# Autodesk Inventor assembly: one side of drive
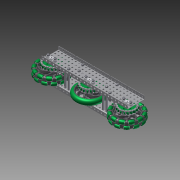
[picture p0: Inventor's stored thumbnail of the model, 180x180]
Saved by Autodesk Inventor 2014 SP1 (Build 180222100, 222)
## iProperties
Created: 2013-08-29
Part Number: one side of drive
Document SubType Name: Assembly
Designer: Ryan
Sending System: SolidWorks 2013
Last Author: Ryan
Author: Ryan
## Documents named in this file (15)
- C:\Users\Ryan\Desktop\sw\toss up 1st A bot\inventor drive\one side of drive.iam
- C:\Users\Ryan\Desktop\sw\lib\Aperture VEX CAD Library\Metal\C Channel\5 x 25.ipt
- C:\Users\Ryan\Desktop\sw\lib\Aperture VEX CAD Library\Bearing Blocks\Bearing Block.ipt
- C:\Users\Ryan\Desktop\sw\lib\Aperture VEX CAD Library\Shaft\2 inch Shaft.ipt
- C:\Users\Ryan\Desktop\sw\toss up 1st A bot\inventor drive\tensioner.iam
- C:\Users\Ryan\Desktop\sw\lib\Aperture VEX CAD Library\Standoffs\BEAM-2000.ipt
- C:\Users\Ryan\Desktop\sw\lib\Aperture VEX CAD Library\Hardware\8-32\8-32 Nylock.ipt
- C:\Users\Ryan\Desktop\sw\lib\Aperture VEX CAD Library\Hardware\8-32\8-32_.500.ipt
- C:\Users\Ryan\Desktop\sw\toss up 1st A bot\inventor drive\wheel assembly.iam
- C:\Users\Ryan\Desktop\sw\lib\Super Sonic Sparks VEX CAD Library\Wheels\4'' (Diameter) Wheel With High Traction Tire.iam
- C:\Users\Ryan\Desktop\sw\lib\Aperture VEX CAD Library\Hardware\Shaft Collar.ipt
- C:\Users\Ryan\Desktop\sw\lib\Aperture VEX CAD Library\Spacers\SPACER-0500-0125.ipt
- C:\Users\Ryan\Desktop\sw\lib\Aperture VEX CAD Library\Sprockets\green\High Strength 18-Tooth Sprocket.ipt
- C:\Users\Ryan\Desktop\sw\toss up 1st A bot\inventor drive\one side of drive\Design Accelerator\V-Belt transmission1.iam
- C:\Users\Ryan\Desktop\sw\lib\Aperture VEX CAD Library\Sprockets\HS Sprockets\High strength Chain Link.ipt
## Components (143 placed, 17 different names)
1. 5 x 25:1 — Mate:1, Mate:2, Mate:3, Mate:4, Mate:63, Mate:64, Angle:1
2. 2 inch shaft:2 — Flush:1, Mate:96, Mate:97
3. 5 x 25:4 — Mate:9, Mate:10, Mate:11, Mate:12, Mate:13, Mate:14, Mate:15, Mate:16, Mate:17, Mate:22, Mate:30, Mate:31, Mate:40, Mate:43, Mate:51, Mate:52, Mate:53, Mate:68, Mate:69, Mate:70, Mate:71, Mate:76, Mate:79, Mate:80, Mate:83, Mate:84, Mate:85, Mate:86, Mate:87, Mate:88, Mate:89, Mate:90, Mate:91
4. 18 tooth hs sprocket:2 — Mate:92, Mate:93, Mate:94, Mate:95, Mate:96, Mate:97, Mate:98
5. tensioner:1 [sub-assembly] — Mate:83, Mate:84, Mate:85
6. tensioner:2 [sub-assembly] — Mate:89, Mate:90, Mate:91
7. tensioner:3 [sub-assembly] — Mate:86, Mate:87, Mate:88
8. tensioner:4 [sub-assembly] — Mate:9, Mate:10, Mate:11
9. tensioner:5 [sub-assembly] — Mate:12, Mate:13, Mate:14, Tangent:1
10. tensioner:6 [sub-assembly] — Mate:15, Mate:16, Mate:17
11. 8-32 nylock:1 — Mate:40
12. 8-32 nylock:2 — Mate:43
13. wheel assembly:1 [sub-assembly] — Mate:67, Mate:68
14. wheel assembly:2 [sub-assembly] — Mate:69, Mate:70, Mate:71
15. 4'' (Diameter) Wheel With High Traction Tire:1 [sub-assembly] — Mate:75
16. Shaft Collar:1 — Mate:75, Mate:92, Mate:95
17. SPACER-0500-0125:1 — Mate:76, Mate:79, Mate:80, Mate:93, Mate:94
18. V-Belt transmission:1 [sub-assembly]
19. bearing block:8 — Mate:30, Mate:31, Mate:52, Mate:56, Mate:57, Mate:67
20. 8-32 nylock:7 — Mate:54, Mate:56
21. 8-32_-375:16 — Mate:51, Mate:54
22. 8-32_-375:17 — Mate:53, Mate:55
23. 8-32 nylock:6 — Mate:55, Mate:57
24. 8-32 nylock:9 — Mate:64, Mate:66
25. 8-32_-375:2 — Mate:66
26. bearing block:1 — Mate:1, Mate:2, Mate:3, Mate:4
27. 8-32_-375:1 — Mate:65
28. 8-32 nylock:8 — Mate:63, Mate:65
29. Bearing Block:5 — Flush:1
30. 8-32 nylock:10
31. 8-32_.500:31
32. 8-32_.500:32
33. 8-32 nylock:11
34. 8-32 nylock:12
35. 8-32_.500:33
36. Bearing Block:6
37. 8-32_.500:34
38. 8-32 nylock:13
39. Bearing Block:7
40. 8-32 nylock:14
41. 8-32_.500:35
42. 8-32_.500:36
43. 8-32 nylock:15
44. 8-32 nylock:16
45. 8-32_.500:37
46. Bearing Block:9
47. 8-32_.500:38
48. 8-32 nylock:17
49. High strength Chain Link:1 — Tangent:1, Mate:98, Angle:1
50. High strength Chain Link:2
51. High strength Chain Link:3
52. High strength Chain Link:4
53. High strength Chain Link:5
54. High strength Chain Link:6
55. High strength Chain Link:7
56. High strength Chain Link:8
57. High strength Chain Link:9
58. High strength Chain Link:10
59. High strength Chain Link:11
60. High strength Chain Link:12
61. High strength Chain Link:13
62. High strength Chain Link:14
63. High strength Chain Link:15
64. High strength Chain Link:16
65. High strength Chain Link:17
66. High strength Chain Link:18
67. High strength Chain Link:19
68. High strength Chain Link:20
69. High strength Chain Link:21
70. High strength Chain Link:22
71. High strength Chain Link:23
72. High strength Chain Link:24
73. High strength Chain Link:25
74. High strength Chain Link:26
75. High strength Chain Link:27
76. High strength Chain Link:28
77. High strength Chain Link:29
78. High strength Chain Link:30
79. High strength Chain Link:31
80. High strength Chain Link:32
81. High strength Chain Link:33
82. High strength Chain Link:34
83. High strength Chain Link:35
84. High strength Chain Link:36
85. High strength Chain Link:37
86. High strength Chain Link:38
87. High strength Chain Link:39
88. High strength Chain Link:40
89. High strength Chain Link:41
90. High strength Chain Link:42
91. High strength Chain Link:43
92. High strength Chain Link:44
93. High strength Chain Link:45
94. High strength Chain Link:46
95. High strength Chain Link:47
96. High strength Chain Link:48
97. High strength Chain Link:49
98. High strength Chain Link:50
99. High strength Chain Link:51
100. High strength Chain Link:52
101. High strength Chain Link:53
102. High strength Chain Link:54
103. High strength Chain Link:55
104. High strength Chain Link:56
105. High strength Chain Link:57
106. High strength Chain Link:58
107. High strength Chain Link:59
108. High strength Chain Link:60
109. High strength Chain Link:61
110. High strength Chain Link:62
111. High strength Chain Link:63
112. High strength Chain Link:64
113. High strength Chain Link:65
114. High strength Chain Link:66
115. High strength Chain Link:67
116. High strength Chain Link:68
117. High strength Chain Link:69
118. High strength Chain Link:70
119. High strength Chain Link:71
120. High strength Chain Link:72
121. High strength Chain Link:73
122. High strength Chain Link:74
123. High strength Chain Link:75
124. High strength Chain Link:76
125. High strength Chain Link:77
126. High strength Chain Link:78
127. High strength Chain Link:79
128. High strength Chain Link:80
129. High strength Chain Link:81
130. High strength Chain Link:82
131. High strength Chain Link:83
132. beam-2000:3 — Mate:22
133. 8-32_-375:29
134. 8-32_-375:26
135. BEAM-2000:4
136. 8-32_.500:28
137. 8-32_.500:30
138. BEAM-2000:5
139. 8-32_.500:39
140. 8-32_.500:40
141. BEAM-2000:6
142. 8-32_.500:41
143. 8-32_.500:42
## Component patterns: (3 elements, first: bearing block:8 + 8-32 nylock:7 + 8-32_-375:16 + 8-32_-375:17 + 8-32 nylock:6 + 8-32 nylock:9 + 8-32_-375:2 + bearing block:1 + 8-32_-375:1 + 8-32 nylock:8), (2 elements), (83 elements, first: High strength Chain Link:1), (2 elements, first: beam-2000:3 + 8-32_-375:29 + 8-32_-375:26), Component Pattern 1:2 (2 elements)
## Relationships (70: Mate 67, Flush 1, Tangent 1, Angle 1)
- Mate:1 (2.3114 mm): 5 x 25:1 ↔ bearing block:1
- Mate:2: 5 x 25:1 ↔ bearing block:1
- Mate:3 (2.3114 mm): 5 x 25:1 ↔ bearing block:1
- Mate:4 (2.3114 mm): 5 x 25:1 ↔ bearing block:1
- [Mate]: bearing block:1 ↔ 8-32_-375:1
- [Mate]: bearing block:1 ↔ 8-32_-375:1
- [Mate]: 8-32_-375:2 ↔ bearing block:1
- [Mate]: 8-32_-375:2 ↔ bearing block:1
- Mate:9 (2.3114 mm): 5 x 25:4 ↔ tensioner:4
- Mate:10 (2.3114 mm): 5 x 25:4 ↔ tensioner:4
- Mate:11: 5 x 25:4 ↔ tensioner:4
- Mate:12 (2.3114 mm): 5 x 25:4 ↔ tensioner:5
- Mate:13 (2.3114 mm): 5 x 25:4 ↔ tensioner:5
- Mate:14: 5 x 25:4 ↔ tensioner:5
- Mate:15 (2.3114 mm): 5 x 25:4 ↔ tensioner:6
- Mate:16 (2.3114 mm): 5 x 25:4 ↔ tensioner:6
- Mate:17: 5 x 25:4 ↔ tensioner:6
- [Mate] (2.3114 mm): 5 x 25:4 ↔ 8-32_-375:26
- [Mate] (2.3114 mm): 5 x 25:4 ↔ 8-32_-375:26
- [Mate]: 5 x 25:4 ↔ 8-32_-375:26
- [Mate]: beam-2000:3 ↔ 8-32_-375:26
- Mate:22: 5 x 25:4 ↔ beam-2000:3
- [Mate]: beam-2000:3 ↔ 8-32_-375:29
- [Mate]: 5 x 25:1 ↔ 8-32_-375:29
- [Mate]: bearing block:8 ↔ 8-32_-375:17
- [Mate]: bearing block:8 ↔ 8-32_-375:16
- Mate:30 (2.3114 mm): 5 x 25:4 ↔ bearing block:8
- Mate:31 (2.3114 mm): 5 x 25:4 ↔ bearing block:8
- [Mate] (2.3114 mm): 5 x 25:4 ↔ 8-32_-375:16
- Mate:40: 5 x 25:4 ↔ 8-32 nylock:1
- Mate:43: 5 x 25:4 ↔ 8-32 nylock:2
- Mate:51: 5 x 25:4 ↔ 8-32_-375:16
- Mate:52: 5 x 25:4 ↔ bearing block:8
- Mate:53: 5 x 25:4 ↔ 8-32_-375:17
- Mate:54: 8-32 nylock:7 ↔ 8-32_-375:16
- Mate:55: 8-32_-375:17 ↔ 8-32 nylock:6
- Mate:56: bearing block:8 ↔ 8-32 nylock:7
- Mate:57: bearing block:8 ↔ 8-32 nylock:6
- Mate:63: 5 x 25:1 ↔ 8-32 nylock:8
- Mate:64: 5 x 25:1 ↔ 8-32 nylock:9
- Mate:65: 8-32_-375:1 ↔ 8-32 nylock:8
- Mate:66: 8-32 nylock:9 ↔ 8-32_-375:2
- Mate:67: wheel assembly:1 ↔ bearing block:8
- Mate:68: 5 x 25:4 ↔ wheel assembly:1
- Mate:69: 5 x 25:4 ↔ wheel assembly:2
- Mate:70 (2.3114 mm): 5 x 25:4 ↔ wheel assembly:2
- Mate:71 (2.3114 mm): 5 x 25:4 ↔ wheel assembly:2
- Mate:75: 4'' (Diameter) Wheel With High Traction Tire:1 ↔ Shaft Collar:1
- Mate:76: 5 x 25:4 ↔ SPACER-0500-0125:1
- Mate:79 (2.3114 mm): 5 x 25:4 ↔ SPACER-0500-0125:1
- Mate:80 (2.3114 mm): 5 x 25:4 ↔ SPACER-0500-0125:1
- Flush:1 (3.175 mm): 2 inch shaft:2 ↔ Bearing Block:5
- Mate:83 (2.3114 mm): 5 x 25:4 ↔ tensioner:1
- Mate:84 (2.3114 mm): 5 x 25:4 ↔ tensioner:1
- Mate:85: 5 x 25:4 ↔ tensioner:1
- Mate:86 (2.3114 mm): 5 x 25:4 ↔ tensioner:3
- Mate:87 (2.3114 mm): 5 x 25:4 ↔ tensioner:3
- Mate:88: 5 x 25:4 ↔ tensioner:3
- Mate:89 (2.3114 mm): 5 x 25:4 ↔ tensioner:2
- Mate:90 (2.3114 mm): 5 x 25:4 ↔ tensioner:2
- Mate:91: 5 x 25:4 ↔ tensioner:2
- Mate:92: 18 tooth hs sprocket:2 ↔ Shaft Collar:1
- Mate:93: 18 tooth hs sprocket:2 ↔ SPACER-0500-0125:1
- Mate:94: 18 tooth hs sprocket:2 ↔ SPACER-0500-0125:1
- Mate:95: 18 tooth hs sprocket:2 ↔ Shaft Collar:1
- Mate:96: 2 inch shaft:2 ↔ 18 tooth hs sprocket:2
- Mate:97: 2 inch shaft:2 ↔ 18 tooth hs sprocket:2
- Tangent:1: tensioner:5 ↔ High strength Chain Link:1
- Mate:98: 18 tooth hs sprocket:2 ↔ High strength Chain Link:1
- Angle:1 (165 deg): 5 x 25:1 ↔ High strength Chain Link:1
## Named parameters: q = 2.3114 mm
